# Autodesk Inventor assembly: motor_ass
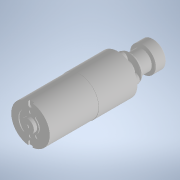
[picture p0: Inventor's stored thumbnail of the model, 180x180]
Saved by Autodesk Inventor 2020 (Build 240168000, 168)
## iProperties
Created: 2019-05-07
Part Number: motor_ass
Document SubType Name: Assembly
Designer: psrob
Author: psrob
## Documents named in this file (3)
- E:\projects-2\project dog gen2\hardware\motor_ass.iam
- E:\projects-2\project dog gen2\hardware\motor_2.ipt
- E:\projects-2\project dog gen2\hardware\2GT_wheel_5.ipt
## Components (2 placed, 2 different names)
1. motor_2:1 — Insert:1
2. 2GT_wheel_5:1 — Insert:1
## Relationships (1: Insert 1)
- Insert:1 (-2 mm): motor_2:1 ↔ 2GT_wheel_5:1
